# Autodesk Inventor assembly: Speleofox PCB 1
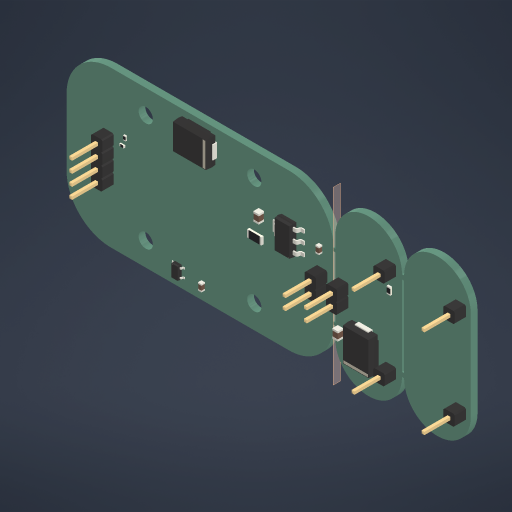
[picture p0: Inventor's stored thumbnail of the model, 512x512]
Saved by Autodesk Inventor 2024 (Build 280153000, 153)
## iProperties
Company: Kicad
Created: 2026-08-19
Part Number: Speleofox PCB 1
Description: KiCad electronic assembly
Document SubType Name: Assembly
Designer: schar
Authority: Unknown
Title: Speleofox PCB.step
Author: Pcbnew
Sending System: KiCad to STEP converter
Preprocessor: Open CASCADE STEP processor 7.9
## Documents named in this file (13)
- C:\Users\schar\Projects\SpeleoFox\cad\Speleofox PCB\Speleofox PCB.iam
- C:\Users\schar\Projects\SpeleoFox\cad\Speleofox PCB\TSOT-23-5.ipt
- C:\Users\schar\Projects\SpeleoFox\cad\Speleofox PCB\D_SMC.ipt
- C:\Users\schar\Projects\SpeleoFox\cad\Speleofox PCB\R_0402_1005Metric.ipt
- C:\Users\schar\Projects\SpeleoFox\cad\Speleofox PCB\PinHeader_1x01_P2.54mm_Vertical.ipt
- C:\Users\schar\Projects\SpeleoFox\cad\Speleofox PCB\C_0603_1608Metric.ipt
- C:\Users\schar\Projects\SpeleoFox\cad\Speleofox PCB\PinHeader_1x02_P2.54mm_Vertical.ipt
- C:\Users\schar\Projects\SpeleoFox\cad\Speleofox PCB\R_1206_3216Metric.ipt
- C:\Users\schar\Projects\SpeleoFox\cad\Speleofox PCB\Fuse_0603_1608Metric.ipt
- C:\Users\schar\Projects\SpeleoFox\cad\Speleofox PCB\SOT-223.ipt
- C:\Users\schar\Projects\SpeleoFox\cad\Speleofox PCB\PinHeader_1x04_P2.54mm_Vertical.ipt
- C:\Users\schar\Projects\SpeleoFox\cad\Speleofox PCB\C_0805_2012Metric.ipt
- C:\Users\schar\Projects\SpeleoFox\cad\Speleofox PCB\SpeleoFox_PCB.ipt
## Components (20 placed, 20 different names)
1. 1
2. 2
3. 3
4. 4
5. 5
6. 6
7. 7
8. 8
9. 9
10. 10
11. 11
12. 12
13. 13
14. 14
15. 15
16. 16
17. 17
18. 18
19. 19
20. 20 — Flush:1
## Relationships (1: Flush 1)
- Flush:1: 20
